# Autodesk Inventor assembly: Door
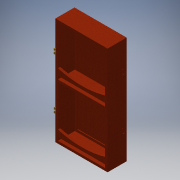
[picture p0: Inventor's stored thumbnail of the model, 180x180]
Saved by Autodesk Inventor 2016 (Build 200138000, 138)
## iProperties
Created: 2017-10-31
Part Number: Door
Document SubType Name: Assembly
Designer: mathaetaes
Author: mathaetaes
## Documents named in this file (9)
- E:\Projects\3D Printer\printer projects\My Designs\Bar Cabinet\Door.iam
- E:\Projects\3D Printer\printer projects\My Designs\Bar Cabinet\Door Side.ipt
- E:\Projects\3D Printer\printer projects\My Designs\Bar Cabinet\Door top.ipt
- E:\Projects\3D Printer\printer projects\My Designs\Bar Cabinet\Door retention wall.ipt
- E:\Projects\3D Printer\printer projects\My Designs\Bar Cabinet\Door Shelf.ipt
- E:\Projects\3D Printer\printer projects\My Designs\Bar Cabinet\Cabinet Moulding Long.ipt
- E:\Projects\3D Printer\printer projects\My Designs\Bar Cabinet\Cabinet Moulding Short.ipt
- E:\Projects\3D Printer\printer projects\My Designs\Bar Cabinet\Door moulding slide-in panel.ipt
- E:\Projects\3D Printer\printer projects\My Designs\Bar Cabinet\hinge left.ipt
## Components (14 placed, 8 different names)
1. Door Side:2 — Mate:9, Mate:12, Flush:15, Flush:16, Flush:21, Flush:22, Mate:22, Mate:23, Mate:24, Mate:25, Mate:26, Mate:27
2. Door retention wall:1 — Flush:12, Mate:7, Mate:15, Flush:21
3. Door Side:3 — Flush:12, Mate:7, Mate:8, Flush:13, Mate:11, Flush:14, Mate:13, Flush:17, Mate:14, Flush:18, Flush:19, Flush:20, Flush:23
4. Door Shelf:1 — Mate:8, Mate:9, Flush:13, Mate:10
5. Door retention wall:2 — Mate:10, Mate:11, Flush:14
6. Door top:2 — Mate:12, Flush:15, Flush:16, Mate:13, Flush:17, Mate:15, Flush:20
7. Door top:3 — Mate:14, Flush:18, Flush:19, Flush:30, Mate:21
8. Cabinet Moulding Long:2 — Flush:23, Flush:24, Flush:25, Flush:26, Mate:16, Flush:27, Flush:28, Mate:17, Flush:29, Flush:30, Mate:18, Mate:21
9. Cabinet Moulding Long:3 — Flush:22, Flush:24, Flush:25, Mate:20
10. Cabinet Moulding Short:1 — Flush:26, Mate:16, Flush:27
11. Cabinet Moulding Short:2 — Flush:28, Mate:17, Flush:29, Mate:19
12. Door moulding slide-in panel:1 — Mate:18, Mate:19, Mate:20
13. hinge left:1 — Mate:22, Mate:23, Mate:24
14. hinge left:2 — Mate:25, Mate:26, Mate:27
## Relationships (40: Mate 21, Flush 19)
- Flush:12: Door retention wall:1 ↔ Door Side:3
- Mate:7: Door retention wall:1 ↔ Door Side:3
- Mate:8: Door Side:3 ↔ Door Shelf:1
- Mate:9: Door Side:2 ↔ Door Shelf:1
- Flush:13: Door Side:3 ↔ Door Shelf:1
- Mate:10 (25.4 mm): Door Shelf:1 ↔ Door retention wall:2
- Mate:11: Door Side:3 ↔ Door retention wall:2
- Flush:14: Door Side:3 ↔ Door retention wall:2
- Mate:12: Door Side:2 ↔ Door top:2
- Flush:15: Door Side:2 ↔ Door top:2
- Flush:16: Door Side:2 ↔ Door top:2
- Mate:13: Door Side:3 ↔ Door top:2
- Flush:17: Door Side:3 ↔ Door top:2
- Mate:14: Door Side:3 ↔ Door top:3
- Flush:18: Door Side:3 ↔ Door top:3
- Flush:19: Door Side:3 ↔ Door top:3
- Mate:15 (25.4 mm): Door retention wall:1 ↔ Door top:2
- Flush:20: Door Side:3 ↔ Door top:2
- Flush:21: Door Side:2 ↔ Door retention wall:1
- Flush:22: Door Side:2 ↔ Cabinet Moulding Long:3
- Flush:23: Door Side:3 ↔ Cabinet Moulding Long:2
- Flush:24: Cabinet Moulding Long:2 ↔ Cabinet Moulding Long:3
- Flush:25: Cabinet Moulding Long:2 ↔ Cabinet Moulding Long:3
- Flush:26: Cabinet Moulding Long:2 ↔ Cabinet Moulding Short:1
- Mate:16: Cabinet Moulding Long:2 ↔ Cabinet Moulding Short:1
- Flush:27: Cabinet Moulding Long:2 ↔ Cabinet Moulding Short:1
- Flush:28: Cabinet Moulding Long:2 ↔ Cabinet Moulding Short:2
- Mate:17: Cabinet Moulding Long:2 ↔ Cabinet Moulding Short:2
- Flush:29: Cabinet Moulding Long:2 ↔ Cabinet Moulding Short:2
- Flush:30: Door top:3 ↔ Cabinet Moulding Long:2
- Mate:18: Cabinet Moulding Long:2 ↔ Door moulding slide-in panel:1
- Mate:19: Cabinet Moulding Short:2 ↔ Door moulding slide-in panel:1
- Mate:20: Cabinet Moulding Long:3 ↔ Door moulding slide-in panel:1
- Mate:21: Door top:3 ↔ Cabinet Moulding Long:2
- Mate:22: Door Side:2 ↔ hinge left:1
- Mate:23: Door Side:2 ↔ hinge left:1
- Mate:24: Door Side:2 ↔ hinge left:1
- Mate:25: Door Side:2 ↔ hinge left:2
- Mate:26: Door Side:2 ↔ hinge left:2
- Mate:27: Door Side:2 ↔ hinge left:2
